# Autodesk Inventor assembly: X_CarriageR_V2_1
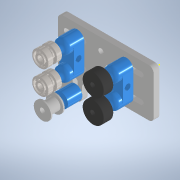
[picture p0: Inventor's stored thumbnail of the model, 180x180]
Saved by Autodesk Inventor 2021 (Build 250183000, 183)
## iProperties
Created: 2021-06-13
Part Number: X_CarriageR_V2_1
Document SubType Name: Assembly
Designer: Jorian Brusind
Author: Jorian Brusind
## Documents named in this file (7)
- C:\Users\Jorian Brusind\Documents\GitHub\PersonalProjects\HyperRail\Inventor Files\X_CarriageR_V2_1.iam
- C:\Users\Jorian Brusind\Documents\GitHub\PersonalProjects\HyperRail\Inventor Files\X_Carriage_Plate.ipt
- C:\Users\Jorian Brusind\Documents\GitHub\PersonalProjects\HyperRail\Inventor Files\Rollder_Spacer_Single.ipt
- C:\Users\Jorian Brusind\Documents\GitHub\PersonalProjects\HyperRail\Inventor Files\10mm_Idle_Pulley.ipt
- C:\Users\Jorian Brusind\Documents\GitHub\PersonalProjects\HyperRail\Inventor Files\4mm_Roller_Spacer_extended.ipt
- C:\Users\Jorian Brusind\Documents\GitHub\PersonalProjects\HyperRail\Inventor Files\11mm_BearingWheel.ipt
- C:\Users\Jorian Brusind\Documents\GitHub\PersonalProjects\HyperRail\Inventor Files\606zz_bearing.ipt
## Components (11 placed, 6 different names)
1. X_Carriage_Plate:1 — Mate:35, Mate:67, Mate:69, Mate:72, Mate:84, Mate:85, Angle:1, Angle:2
2. Rollder_Spacer_Single:1 — Mate:35, Mate:40, Mate:42, Mate:67
3. 10mm_Idle_Pulley:1 — Mate:40, Mate:42
4. 4mm_Roller_Spacer_extended:1 — Mate:72, Mate:74, Mate:75, Mate:76, Mate:85, Angle:1
5. 4mm_Roller_Spacer_extended:3 — Mate:69, Mate:81, Mate:82, Mate:83, Mate:84, Angle:2
6. 11mm_BearingWheel:1 — Mate:75, Flush:1, Mate:76
7. 11mm_BearingWheel:2 — Mate:74, Flush:1
8. 606zz_bearing:1 — Mate:82, Flush:2
9. 606zz_bearing:2
10. 606zz_bearing:3 — Mate:81, Flush:2
11. 606zz_bearing:4 — Mate:83
## Relationships (22: Mate 18, Flush 2, Angle 2)
- Mate:35: X_Carriage_Plate:1 ↔ Rollder_Spacer_Single:1
- Mate:40: Rollder_Spacer_Single:1 ↔ 10mm_Idle_Pulley:1
- Mate:42: Rollder_Spacer_Single:1 ↔ 10mm_Idle_Pulley:1
- Mate:67 (-18 mm): X_Carriage_Plate:1 ↔ Rollder_Spacer_Single:1
- Mate:69: X_Carriage_Plate:1 ↔ 4mm_Roller_Spacer_extended:3
- Mate:72: X_Carriage_Plate:1 ↔ 4mm_Roller_Spacer_extended:1
- Mate:74: 4mm_Roller_Spacer_extended:1 ↔ 11mm_BearingWheel:2
- Mate:75: 4mm_Roller_Spacer_extended:1 ↔ 11mm_BearingWheel:1
- Flush:1: 11mm_BearingWheel:1 ↔ 11mm_BearingWheel:2
- Mate:76: 4mm_Roller_Spacer_extended:1 ↔ 11mm_BearingWheel:1
- [Mate]: 606zz_bearing:1 ↔ 606zz_bearing:2
- [Mate] (3 mm): 606zz_bearing:1 ↔ 606zz_bearing:2
- [Mate]: 606zz_bearing:3 ↔ 606zz_bearing:4
- [Mate] (3 mm): 606zz_bearing:3 ↔ 606zz_bearing:4
- Mate:81: 4mm_Roller_Spacer_extended:3 ↔ 606zz_bearing:3
- Mate:82: 4mm_Roller_Spacer_extended:3 ↔ 606zz_bearing:1
- Flush:2: 606zz_bearing:1 ↔ 606zz_bearing:3
- Mate:83: 4mm_Roller_Spacer_extended:3 ↔ 606zz_bearing:4
- Mate:84 (-12.5 mm): X_Carriage_Plate:1 ↔ 4mm_Roller_Spacer_extended:3
- Mate:85 (-12.5 mm): X_Carriage_Plate:1 ↔ 4mm_Roller_Spacer_extended:1
- Angle:1 (0 deg): X_Carriage_Plate:1 ↔ 4mm_Roller_Spacer_extended:1
- Angle:2 (0 deg): X_Carriage_Plate:1 ↔ 4mm_Roller_Spacer_extended:3
## Named parameters: d119_d83 = 0 mm, d120_d85 = 3 mm
